# Autodesk Inventor assembly: 投幣機
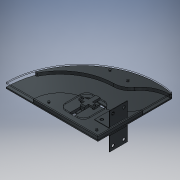
[picture p0: Inventor's stored thumbnail of the model, 180x180]
Saved by Autodesk Inventor 2017 (Build 210142000, 142)
## iProperties
Part Number: 投幣機
Material: 一般
Document SubType Name: Assembly
Designer: G
Author: G
## Documents named in this file (6)
- \\MissGAME-NAS\Miss GAME\松菸-幻影光靈\機關\投幣機\投幣機.iam
- \\MissGAME-NAS\Miss GAME\松菸-幻影光靈\機關\投幣機\實體1.ipt
- \\MissGAME-NAS\Miss GAME\松菸-幻影光靈\機關\投幣機\實體4.ipt
- \\MissGAME-NAS\Miss GAME\松菸-幻影光靈\機關\投幣機\實體5.ipt
- \\MissGAME-NAS\Miss GAME\松菸-幻影光靈\機關\武器把手\RX672-NW.ipt
- \\MissGAME-NAS\Miss GAME\模型庫\L固定板_25x30.ipt
## Components (7 placed, 5 different names)
1. 實體1:1 — 齊平:1, 齊平:2, 貼合:1, 齊平:3
2. 實體4:1 — 插入:1, 插入:2
3. 實體5:1 — 貼合:2
4. 實體5:2 — 插入:1, 插入:2, 貼合:3
5. RX672-NW:1 — 齊平:1, 齊平:2, 貼合:1
6. L固定板_25x30:1 — 齊平:3, 貼合:2, 齊平:4, 齊平:5
7. L固定板_25x30:2 — 齊平:4, 貼合:3, 齊平:5
## Relationships (10: Flush 5, Mate 3, Insert 2)
- 插入:1 [Insert]: 實體4:1 ↔ 實體5:2
- 插入:2 [Insert]: 實體4:1 ↔ 實體5:2
- 齊平:1 [Flush]: 實體1:1 ↔ RX672-NW:1
- 齊平:2 [Flush]: 實體1:1 ↔ RX672-NW:1
- 貼合:1 [Mate] (0.5 mm): 實體1:1 ↔ RX672-NW:1
- 齊平:3 [Flush]: 實體1:1 ↔ L固定板_25x30:1
- 貼合:2 [Mate]: 實體5:1 ↔ L固定板_25x30:1
- 齊平:4 [Flush]: L固定板_25x30:1 ↔ L固定板_25x30:2
- 貼合:3 [Mate]: 實體5:2 ↔ L固定板_25x30:2
- 齊平:5 [Flush]: L固定板_25x30:1 ↔ L固定板_25x30:2
